# Autodesk Inventor assembly: California_Corner
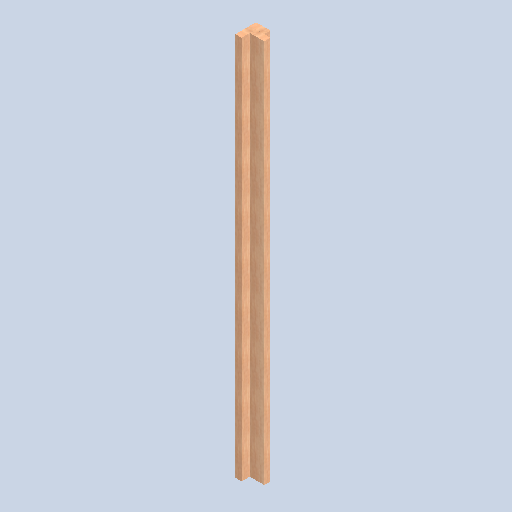
[picture p0: Inventor's stored thumbnail of the model, 512x512]
Saved by Autodesk Inventor 2025 (Build 290162010, 162A)
## iProperties
Created: 2024-09-15
Part Number: California_Corner
Document SubType Name: Assembly
Designer: Tom
Author: Tom
## Documents named in this file (2)
- C:\Users\Tom\Documents\Inventor\Mobility\Additional_Building\California_Corner.iam
- C:\Users\Tom\Documents\Inventor\Mobility\Additional_Building\Stud_With_Height_93_Inches.ipt
## Components (3 placed, 1 different names)
1. Stud_With_Height_93_Inches:1 — Mate:1, Flush:1, Flush:2, Mate:3, Flush:3
2. Stud_With_Height_93_Inches:2 — Mate:1, Flush:1, Flush:2, Mate:2
3. Stud_With_Height_93_Inches:3 — Mate:2, Mate:3, Flush:3
## Relationships (6: Mate 3, Flush 3)
- Mate:1: Stud_With_Height_93_Inches:1 ↔ Stud_With_Height_93_Inches:2
- Flush:1: Stud_With_Height_93_Inches:1 ↔ Stud_With_Height_93_Inches:2
- Flush:2: Stud_With_Height_93_Inches:1 ↔ Stud_With_Height_93_Inches:2
- Mate:2: Stud_With_Height_93_Inches:2 ↔ Stud_With_Height_93_Inches:3
- Mate:3: Stud_With_Height_93_Inches:1 ↔ Stud_With_Height_93_Inches:3
- Flush:3: Stud_With_Height_93_Inches:1 ↔ Stud_With_Height_93_Inches:3
